# Autodesk Inventor assembly: WheelAssembly
Saved by Autodesk Inventor 2015 (Build 190159000, 159)
## iProperties
Created: 2015-01-17
Part Number: WheelAssembly
Document SubType Name: Assembly
Designer: jhirshland1
Author: jhirshland1
## Documents named in this file (4)
- C:\Users\jhirshland1\Inventor\HWRobot2015\FRCKOP2015\AndyMark\WheelAssembly.iam
- C:\Users\jhirshland1\Inventor\HWRobot2015\FRCKOP2015\Drive Base\Toughbox Mini L-Base.iam
- C:\Users\jhirshland1\Inventor\HWRobot2015\FRCKOP2015\AndyMark\217-2585.20121203.iam
- C:\Users\jhirshland1\Inventor\HWRobot2015\Imported Components\217-2592-STEP-20140805\217-2592-STEP-20140805.ipt
## Components (4 placed, 3 different names)
1. Toughbox Mini L-Base:1 [sub-assembly]
2. 217-2585.20121203:1 [sub-assembly]
3. 217-2592-STEP-20140805:1
4. 217-2592-STEP-20140805:2
## Relationships (7: Insert 5, Mate 2)
- [Insert]: 217-2585.20121203:1 ↔ 217-2592-STEP-20140805:1
- [Insert]: 217-2585.20121203:1 ↔ 217-2592-STEP-20140805:1
- [Insert]: 217-2585.20121203:1 ↔ 217-2592-STEP-20140805:1
- [Insert]: 217-2585.20121203:1 ↔ 217-2592-STEP-20140805:2
- [Insert]: 217-2585.20121203:1 ↔ 217-2592-STEP-20140805:2
- [Mate]: Toughbox Mini L-Base:1 ↔ 217-2592-STEP-20140805:1
- [Mate]: Toughbox Mini L-Base:1 ↔ 217-2592-STEP-20140805:1
